# Autodesk Inventor assembly: ForeArm
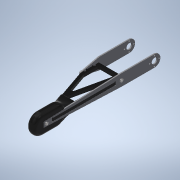
[picture p0: Inventor's stored thumbnail of the model, 180x180]
Saved by Autodesk Inventor 2020.4 (Build 244396000, 396)
## iProperties
Created: 2016-05-04
Part Number: ForeArm
Document SubType Name: Assembly
Designer: hiroaki
Mass: 59.7567 g
Surface Area: 275.043 cm^2
Volume: 46.6042 cm^3
Density: 1.28222 g/cm^3
Author: hiroaki
## Documents named in this file (7)
- C:\Users\Masato\Documents\Inventor\CIT Brains_Inventor\OpenPlatform_ver3_0\UpperBody\Arm\ForeArm.iam
- C:\Users\Masato\Documents\Inventor\CIT Brains_Inventor\OpenPlatform_ver3_0\UpperBody\Arm\ForeArm_vertical_frame02.ipt
- C:\Users\Masato\Documents\Inventor\CIT Brains_Inventor\OpenPlatform_ver3_0\UpperBody\Arm\ForeArm_vertical_frame01.ipt
- C:\Users\Masato\Documents\Inventor\CIT Brains_Inventor\OpenPlatform_ver3_0\UpperBody\Arm\ForeArm_vertical_frame03.ipt
- C:\Users\Masato\Documents\Inventor\CIT Brains_Inventor\OpenPlatform_ver3_0\UpperBody\Arm\Hand.ipt
- C:\Users\Masato\Documents\Inventor\CIT Brains_Inventor\OpenPlatform_ver3_0\Ready_Made\Screw\M3-6.ipt
- C:\Users\Masato\Documents\Inventor\CIT Brains_Inventor\OpenPlatform_ver3_0\Ready_Made\Screw\M3-10.ipt
## Components (8 placed, 6 different names)
1. ForeArm_vertical_frame01:1 — メイト:1, メイト:2, フラッシュ:1, 挿入:3, 挿入:4, 挿入:5, 挿入:6, メイト:4, メイト:5
2. ForeArm_vertical_frame02:1 — 挿入:3, 挿入:4, メイト:3, 挿入:7, 挿入:10
3. ForeArm_vertical_frame03:1 — 挿入:5, 挿入:6, 挿入:8, 挿入:9
4. Hand:1 — メイト:3, メイト:4, メイト:5
5. M3-6:1 — 挿入:7
6. M3-6:2 — 挿入:8
7. M3-6:3 — 挿入:9
8. M3-10:1 — 挿入:10
## Relationships (14: Insert 8, Mate 5, Flush 1)
- メイト:1 [Mate]: ForeArm_vertical_frame01:1
- メイト:2 [Mate]: ForeArm_vertical_frame01:1
- フラッシュ:1 [Flush]: ForeArm_vertical_frame01:1
- 挿入:3 [Insert]: ForeArm_vertical_frame01:1 ↔ ForeArm_vertical_frame02:1
- 挿入:4 [Insert]: ForeArm_vertical_frame01:1 ↔ ForeArm_vertical_frame02:1
- 挿入:5 [Insert]: ForeArm_vertical_frame01:1 ↔ ForeArm_vertical_frame03:1
- 挿入:6 [Insert]: ForeArm_vertical_frame01:1 ↔ ForeArm_vertical_frame03:1
- メイト:3 [Mate]: ForeArm_vertical_frame02:1 ↔ Hand:1
- メイト:4 [Mate]: ForeArm_vertical_frame01:1 ↔ Hand:1
- メイト:5 [Mate]: ForeArm_vertical_frame01:1 ↔ Hand:1
- 挿入:7 [Insert]: ForeArm_vertical_frame02:1 ↔ M3-6:1
- 挿入:8 [Insert]: ForeArm_vertical_frame03:1 ↔ M3-6:2
- 挿入:9 [Insert]: ForeArm_vertical_frame03:1 ↔ M3-6:3
- 挿入:10 [Insert]: ForeArm_vertical_frame02:1 ↔ M3-10:1
